# Autodesk Inventor assembly: IMS-10-000
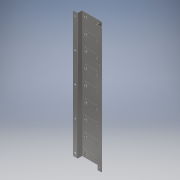
[picture p0: Inventor's stored thumbnail of the model, 180x180]
Saved by Autodesk Inventor 2021 (Build 250183000, 183)
## iProperties
Created: 2020-10-06
Part Number: IMS-10-000
Document SubType Name: Assembly
Designer: mahra
Mass: 4944.25 g
Surface Area: 5566.25 cm^2
Volume: 642.136 cm^3
Density: 7.69969 g/cm^3
Author: mahra
## Documents named in this file (4)
- C:\Users\mahra\Documents\Undervisning\2020-interactive-mech-systems\training-device\IMS-10-000.iam
- C:\Users\mahra\Documents\Undervisning\2020-interactive-mech-systems\training-device\IMS-10-001.ipt
- C:\Users\mahra\Documents\Undervisning\2020-interactive-mech-systems\training-device\IMS-10-002.ipt
- C:\Users\mahra\Documents\CAD\Standard_parts\Fasteners\Welding\DIN929\WLD-NUT_DIN929_M8.ipt
## Components (20 placed, 3 different names)
1. IMS-10-001:1 — Mate:1, Flush:1, Flush:2
2. IMS-10-002:1 — Mate:1, Flush:1, Flush:2, Mate:2, Mate:3, Mate:4, Mate:5
3. WLD-NUT_DIN929_M8:1 — Mate:2, Mate:3
4. WLD-NUT_DIN929_M8:2 — Mate:4, Mate:5
5. WLD-NUT_DIN929_M8:3
6. WLD-NUT_DIN929_M8:4
7. WLD-NUT_DIN929_M8:5
8. WLD-NUT_DIN929_M8:6
9. WLD-NUT_DIN929_M8:7
10. WLD-NUT_DIN929_M8:8
11. WLD-NUT_DIN929_M8:9
12. WLD-NUT_DIN929_M8:10
13. WLD-NUT_DIN929_M8:11
14. WLD-NUT_DIN929_M8:12
15. WLD-NUT_DIN929_M8:13
16. WLD-NUT_DIN929_M8:14
17. WLD-NUT_DIN929_M8:15
18. WLD-NUT_DIN929_M8:16
19. WLD-NUT_DIN929_M8:17
20. WLD-NUT_DIN929_M8:18
## Component patterns: (9 elements, first: WLD-NUT_DIN929_M8:1 + WLD-NUT_DIN929_M8:2)
## Relationships (7: Mate 5, Flush 2)
- Mate:1: IMS-10-001:1 ↔ IMS-10-002:1
- Flush:1 (7.5 mm): IMS-10-001:1 ↔ IMS-10-002:1
- Flush:2 (5 mm): IMS-10-001:1 ↔ IMS-10-002:1
- Mate:2: IMS-10-002:1 ↔ WLD-NUT_DIN929_M8:1
- Mate:3: IMS-10-002:1 ↔ WLD-NUT_DIN929_M8:1
- Mate:4: IMS-10-002:1 ↔ WLD-NUT_DIN929_M8:2
- Mate:5: IMS-10-002:1 ↔ WLD-NUT_DIN929_M8:2
